# Autodesk Inventor assembly: Arm2
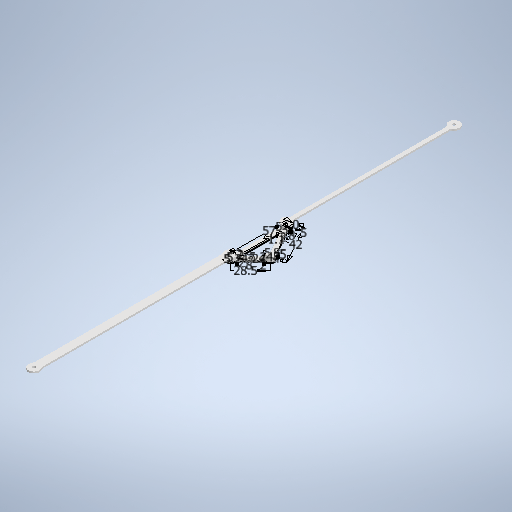
[picture p0: Inventor's stored thumbnail of the model, 512x512]
Saved by Autodesk Inventor 2025.2 (Build 292293000, 293)
## iProperties
Created: 2025-05-22
Part Number: Arm2
Document SubType Name: Assembly
Designer: Admin
Author: Admin
## Documents named in this file (4)
- C:\Users\Admin\Documents\IITD\Robotics\robo arm zen\Arm2.iam
- C:\Users\Admin\Documents\IITD\Robotics\robo arm zen\A2P1.ipt
- C:\Users\Admin\Documents\IITD\Robotics\robo arm zen\A2P2.ipt
- C:\Users\Admin\Documents\IITD\Robotics\robo arm zen\A2P3.ipt
## Components (3 placed, 3 different names)
1. A2P1:1 — Insert:1
2. A2P2:1 — Insert:1, Insert:2
3. A2P3:1 — Insert:2
## Relationships (2: Insert 2)
- Insert:1: A2P1:1 ↔ A2P2:1
- Insert:2: A2P2:1 ↔ A2P3:1
